# Autodesk Inventor assembly: MechanicalHand
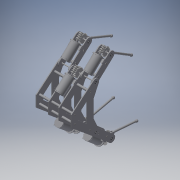
[picture p0: Inventor's stored thumbnail of the model, 180x180]
Saved by Autodesk Inventor 2018 (Build 220112000, 112)
## iProperties
Created: 2017-06-01
Part Number: MechanicalHand
Document SubType Name: Assembly
Designer: Damian
Author: Damian
## Documents named in this file (13)
- C:\Users\Damian\MechanicalHand\CAD\MechanicalHand.iam
- C:\Users\Damian\MechanicalHand\CAD\MechanicalFinger.iam
- C:\Users\Damian\MechanicalHand\CAD\MechanicalPalm.iam
- C:\Users\Damian\MechanicalHand\CAD\EndJoint.ipt
- C:\Users\Damian\MechanicalHand\CAD\LongShaft\LongShaft.ipt
- C:\Users\Damian\MechanicalHand\StandardParts\RetainingRingLarge.ipt
- C:\Users\Damian\MechanicalHand\StandardParts\RetainingRingSmall.ipt
- C:\Users\Damian\MechanicalHand\CAD\MechanicalHand\Design Accelerator\Worm Gears5.iam
- C:\Users\Damian\MechanicalHand\CAD\MechanicalHand\Design Accelerator\Worm Gears6.iam
- C:\Users\Damian\MechanicalHand\CAD\MechanicalHand\Design Accelerator\Worm Gears7.iam
- C:\Users\Damian\MechanicalHand\CAD\MechanicalHand\Design Accelerator\Worm Gears8.iam
- C:\Users\Damian\MechanicalHand\CAD\MechanicalHand\Design Accelerator\Worm Gears9.iam
- C:\Users\Damian\MechanicalHand\CAD\MechanicalHand\Design Accelerator\Worm Gears10.iam
## Components (29 placed, 7 different names)
1. MechanicalFinger:1 [sub-assembly] — Mate:1, Angle:2, Mate:16, Mate:17, Mate:51, Rotation:4, Mate:69, Mate:70
2. MechanicalFinger:2 [sub-assembly] — Mate:8, Angle:1, Mate:12, Mate:13, Mate:57, Mate:65, Mate:66
3. MechanicalFinger:3 [sub-assembly] — Mate:5, Angle:2, Mate:18, Mate:19, Mate:52, Mate:67, Mate:68
4. MechanicalPalm:1 [sub-assembly] — Mate:1, Mate:3, Mate:4, Mate:5, Mate:7, Mate:8, Mate:10, Mate:22, Mate:28, Mate:29, Mate:38, Mate:59, Mate:61
5. MechanicalFinger:4 [sub-assembly] — Mate:10, Angle:1, Mate:14, Mate:15, Mate:58, Rotation:2, Mate:63, Mate:64
6. EndJoint:1 — Mate:16, Mate:17, Rotation:8
7. EndJoint:2 — Mate:18, Mate:19, Rotation:7
8. EndJoint:3 — Mate:12, Mate:13, Rotation:6
9. EndJoint:4 — Mate:14, Mate:15, Rotation:5
10. LongShaft:1 — Mate:28, Mate:29, Mate:30, Mate:31, Mate:32, Mate:33, Mate:34, Mate:35, Mate:36, Mate:37, Mate:53, Mate:54, Mate:55, Mate:56, Mate:60, Rotation:1, Rotation:2
11. LongShaft:2 — Mate:22, Mate:38, Mate:39, Mate:40, Mate:41, Mate:42, Mate:43, Mate:44, Mate:45, Mate:46, Mate:47, Mate:48, Mate:49, Mate:50, Mate:62, Rotation:3, Rotation:4
12. RetainingRingLarge:1 — Mate:30, Mate:32, Angle:3
13. RetainingRingLarge:2 — Mate:31, Mate:33, Angle:3
14. RetainingRingLarge:3 — Mate:39, Mate:48
15. RetainingRingLarge:4 — Mate:40, Mate:47
16. RetainingRingSmall:1 — Mate:34, Mate:54
17. RetainingRingSmall:2 — Mate:35, Mate:53, Mate:58
18. RetainingRingSmall:3 — Mate:36, Mate:55
19. RetainingRingSmall:4 — Mate:37, Mate:56, Mate:57
20. RetainingRingSmall:5 — Mate:42, Mate:46, Mate:52
21. RetainingRingSmall:6 — Mate:41, Mate:45
22. RetainingRingSmall:7 — Mate:44, Mate:49, Mate:51
23. RetainingRingSmall:8 — Mate:43, Mate:50
24. Worm Gears:1 [sub-assembly] — Mate:59, Mate:60, Rotation:1
25. Worm Gears:2 [sub-assembly] — Mate:61, Mate:62, Rotation:3
26. Worm Gears:3 [sub-assembly] — Mate:63, Mate:64, Rotation:5
27. Worm Gears:4 [sub-assembly] — Mate:65, Mate:66, Rotation:6
28. Worm Gears:5 [sub-assembly] — Mate:67, Mate:68, Rotation:7
29. Worm Gears:6 [sub-assembly] — Mate:69, Mate:70, Rotation:8
## Relationships (70: Mate 59, RelateRotation 8, Angle 3)
- Mate:1: MechanicalFinger:1 ↔ MechanicalPalm:1
- Mate:3: MechanicalPalm:1
- Mate:4: MechanicalPalm:1
- Mate:5: MechanicalFinger:3 ↔ MechanicalPalm:1
- Mate:7: MechanicalPalm:1
- Mate:8: MechanicalFinger:2 ↔ MechanicalPalm:1
- Mate:10: MechanicalPalm:1 ↔ MechanicalFinger:4
- Angle:1 (0 deg): MechanicalFinger:2 ↔ MechanicalFinger:4
- Angle:2 (0 deg): MechanicalFinger:1 ↔ MechanicalFinger:3
- Mate:12: MechanicalFinger:2 ↔ EndJoint:3
- Mate:13: MechanicalFinger:2 ↔ EndJoint:3
- Mate:14: MechanicalFinger:4 ↔ EndJoint:4
- Mate:15: MechanicalFinger:4 ↔ EndJoint:4
- Mate:16: MechanicalFinger:1 ↔ EndJoint:1
- Mate:17: MechanicalFinger:1 ↔ EndJoint:1
- Mate:18: MechanicalFinger:3 ↔ EndJoint:2
- Mate:19: MechanicalFinger:3 ↔ EndJoint:2
- Mate:22: MechanicalPalm:1 ↔ LongShaft:2
- Mate:28: MechanicalPalm:1 ↔ LongShaft:1
- Mate:29: MechanicalPalm:1 ↔ LongShaft:1
- Mate:30: LongShaft:1 ↔ RetainingRingLarge:1
- Mate:31: LongShaft:1 ↔ RetainingRingLarge:2
- Mate:32: LongShaft:1 ↔ RetainingRingLarge:1
- Mate:33: LongShaft:1 ↔ RetainingRingLarge:2
- Angle:3 (0 deg): RetainingRingLarge:1 ↔ RetainingRingLarge:2
- Mate:34: LongShaft:1 ↔ RetainingRingSmall:1
- Mate:35: LongShaft:1 ↔ RetainingRingSmall:2
- Mate:36: LongShaft:1 ↔ RetainingRingSmall:3
- Mate:37: LongShaft:1 ↔ RetainingRingSmall:4
- Mate:38: MechanicalPalm:1 ↔ LongShaft:2
- Mate:39: LongShaft:2 ↔ RetainingRingLarge:3
- Mate:40: LongShaft:2 ↔ RetainingRingLarge:4
- Mate:41: LongShaft:2 ↔ RetainingRingSmall:6
- Mate:42: LongShaft:2 ↔ RetainingRingSmall:5
- Mate:43: LongShaft:2 ↔ RetainingRingSmall:8
- Mate:44: LongShaft:2 ↔ RetainingRingSmall:7
- Mate:45: LongShaft:2 ↔ RetainingRingSmall:6
- Mate:46: LongShaft:2 ↔ RetainingRingSmall:5
- Mate:47: LongShaft:2 ↔ RetainingRingLarge:4
- Mate:48: LongShaft:2 ↔ RetainingRingLarge:3
- Mate:49: LongShaft:2 ↔ RetainingRingSmall:7
- Mate:50: LongShaft:2 ↔ RetainingRingSmall:8
- Mate:51: MechanicalFinger:1 ↔ RetainingRingSmall:7
- Mate:52: MechanicalFinger:3 ↔ RetainingRingSmall:5
- Mate:53: LongShaft:1 ↔ RetainingRingSmall:2
- Mate:54: LongShaft:1 ↔ RetainingRingSmall:1
- Mate:55: LongShaft:1 ↔ RetainingRingSmall:3
- Mate:56: LongShaft:1 ↔ RetainingRingSmall:4
- Mate:57: MechanicalFinger:2 ↔ RetainingRingSmall:4
- Mate:58: MechanicalFinger:4 ↔ RetainingRingSmall:2
- Mate:59: MechanicalPalm:1 ↔ Worm Gears:1
- Mate:60: LongShaft:1 ↔ Worm Gears:1
- Mate:61: MechanicalPalm:1 ↔ Worm Gears:2
- Mate:62: LongShaft:2 ↔ Worm Gears:2
- Rotation:1 [RelateRotation] (1 ul): LongShaft:1 ↔ Worm Gears:1
- Rotation:2 [RelateRotation] (1 ul): MechanicalFinger:4 ↔ LongShaft:1
- Rotation:3 [RelateRotation] (1 ul): LongShaft:2 ↔ Worm Gears:2
- Rotation:4 [RelateRotation] (1 ul): MechanicalFinger:1 ↔ LongShaft:2
- Mate:63: MechanicalFinger:4 ↔ Worm Gears:3
- Mate:64: MechanicalFinger:4 ↔ Worm Gears:3
- Rotation:5 [RelateRotation] (1 ul): EndJoint:4 ↔ Worm Gears:3
- Mate:65: MechanicalFinger:2 ↔ Worm Gears:4
- Mate:66: MechanicalFinger:2 ↔ Worm Gears:4
- Rotation:6 [RelateRotation] (1 ul): EndJoint:3 ↔ Worm Gears:4
- Mate:67: MechanicalFinger:3 ↔ Worm Gears:5
- Mate:68: MechanicalFinger:3 ↔ Worm Gears:5
- Rotation:7 [RelateRotation] (1 ul): EndJoint:2 ↔ Worm Gears:5
- Mate:69: MechanicalFinger:1 ↔ Worm Gears:6
- Mate:70: MechanicalFinger:1 ↔ Worm Gears:6
- Rotation:8 [RelateRotation] (1 ul): EndJoint:1 ↔ Worm Gears:6
